# Autodesk Inventor assembly: who_needs_arms
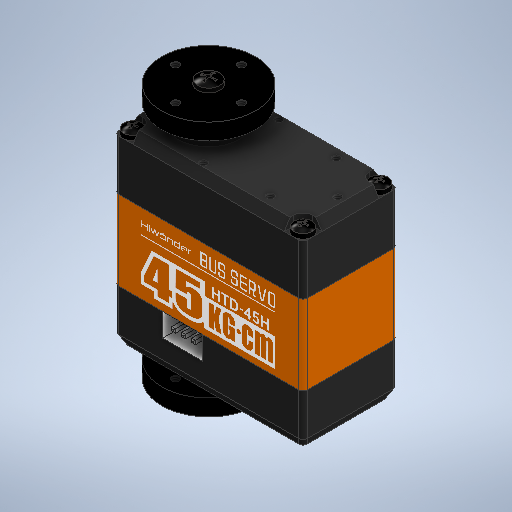
[picture p0: Inventor's stored thumbnail of the model, 512x512]
Saved by Autodesk Inventor 2025.2 (Build 292293000, 293)
## iProperties
Created: 2025-03-25
Part Number: who_needs_arms
Document SubType Name: Assembly
Designer: User
Author: User
## Documents named in this file (2)
- C:\Users\User\Documents\The Maverick's Files\College 3-3\로보인 프로젝트\RHp_hardware_example\Lord Marquaad E\who_needs_arms.iam
- C:\Users\User\Documents\The Maverick's Files\College 3-3\로보인 프로젝트\RHp_hardware_example\Part\HTD-45H, Horn\HTD-45H Assembly.iam
## Components (1 placed, 1 different names)
1. HTD-45H Assembly:1 [sub-assembly] — Flush:2, Flush:1, Flush:3
## Relationships (3: Flush 3)
- Flush:2: HTD-45H Assembly:1
- Flush:1: HTD-45H Assembly:1
- Flush:3: HTD-45H Assembly:1
